# Autodesk Inventor assembly: roller abd rubber purnima samararatne
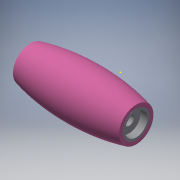
[picture p0: Inventor's stored thumbnail of the model, 180x180]
Saved by Autodesk Inventor 2018 (Build 220112000, 112)
## iProperties
Created: 2017-09-19
Part Number: roller abd rubber purnima samararatne
Document SubType Name: Assembly
Designer: M227958
Author: M227958
## Documents named in this file (3)
- E:\roller abd rubber purnima samararatne.iam
- E:\roller rubber test.ipt
- E:\roller test.ipt
## Components (2 placed, 2 different names)
1. roller rubber test:1 — Mate:1, Mate:2
2. roller test:1 — Mate:1, Mate:2
## Relationships (2: Mate 2)
- Mate:1: roller rubber test:1 ↔ roller test:1
- Mate:2: roller rubber test:1 ↔ roller test:1
